# Autodesk Inventor assembly: Miniature_Steam_Engine
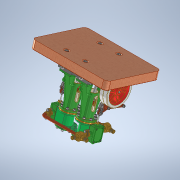
[picture p0: Inventor's stored thumbnail of the model, 180x180]
Saved by Autodesk Inventor 2020 (Build 240168000, 168)
## iProperties
Created: 2023-08-09
Part Number: Miniature_Steam_Engine
Document SubType Name: Assembly
Designer: ACER
Author: ACER
## Documents named in this file (59)
- D:\inventor\bt_tuluyen\ME\Miniature_Steam_Engine.iam
- D:\inventor\bt_tuluyen\ME\Stand_1.ipt
- D:\inventor\bt_tuluyen\ME\Base.ipt
- D:\inventor\bt_tuluyen\ME\Lower_Base_Bearing_Holder_4.ipt
- D:\inventor\bt_tuluyen\ME\Upper_Base_Bearing_Holder_7.ipt
- D:\inventor\bt_tuluyen\ME\Crankshaft.ipt
- D:\inventor\bt_tuluyen\ME\Upper_Base_Bearing_Holder2_8.ipt
- D:\inventor\bt_tuluyen\ME\Assembly_Eccentric.iam
- D:\inventor\bt_tuluyen\ME\Lower_Base_Bearing_Holder2_5.ipt
- D:\inventor\bt_tuluyen\ME\Welding_assembly_Standard.iam
- D:\inventor\bt_tuluyen\ME\Eccentric_rod.ipt
- D:\inventor\bt_tuluyen\ME\Flywhee_l.ipt
- D:\inventor\bt_tuluyen\ME\Bearing_Keeper_11.ipt
- D:\inventor\bt_tuluyen\ME\Conecting_Rod_12.ipt
- D:\inventor\bt_tuluyen\ME\Crankrod_13.ipt
- D:\inventor\bt_tuluyen\ME\Crosshead_14.ipt
- C:\Users\ACER\Documents\Inventor\Content Center Files\R2020\en-US\DIN 128\DIN 128 - A4.ipt
- C:\Users\ACER\Documents\Inventor\Content Center Files\R2020\en-US\DIN 912\DIN 912 - M4 x 0.7 x 30 x 20.ipt
- D:\inventor\bt_tuluyen\ME\Crankrod_Pin_15.ipt
- D:\inventor\bt_tuluyen\ME\Crankrod_Bolt_16.ipt
- D:\inventor\bt_tuluyen\ME\Cylinder_Packnut_18.ipt
- D:\inventor\bt_tuluyen\ME\Cylinder_cover_lower_19.ipt
- D:\inventor\bt_tuluyen\ME\Cylinder_left_.ipt
- D:\inventor\bt_tuluyen\ME\Cylinder_right_.ipt
- D:\inventor\bt_tuluyen\ME\Steam_Piston.ipt
- D:\inventor\bt_tuluyen\ME\Steam_Piston_Ring_.ipt
- D:\inventor\bt_tuluyen\ME\Steam_Piston_Rod_.ipt
- C:\Users\ACER\Documents\Inventor\Content Center Files\R2020\en-US\DIN 934\DIN 934 - M8 x 1.ipt
- D:\inventor\bt_tuluyen\ME\Cylinder_Packing_25.ipt
- D:\inventor\bt_tuluyen\ME\Upper_Cylinder_Cover_26.ipt
- D:\inventor\bt_tuluyen\ME\Assembly_Cylinder_piping_entry_.iam
- D:\inventor\bt_tuluyen\ME\Assembly_Cylinder_Piping_Exit_.iam
- D:\inventor\bt_tuluyen\ME\Valve_Plate_.ipt
- D:\inventor\bt_tuluyen\ME\Steamchest_.ipt
- D:\inventor\bt_tuluyen\ME\Valvel_Packnut_.ipt
- D:\inventor\bt_tuluyen\ME\Slide_Valve_.ipt
- D:\inventor\bt_tuluyen\ME\Side_Valve_Holder_.ipt
- D:\inventor\bt_tuluyen\ME\Steam_chest_slide_value_rod_.ipt
- D:\inventor\bt_tuluyen\ME\Steamchest_cover_.ipt
- D:\inventor\bt_tuluyen\ME\Reverse_Gear_Link_.ipt
- D:\inventor\bt_tuluyen\ME\Revert_Gear_Lever_God_.ipt
- D:\inventor\bt_tuluyen\ME\Reverse_gear_lever_.ipt
- D:\inventor\bt_tuluyen\ME\Revert_gear_level_link_pt.ipt
- D:\inventor\bt_tuluyen\ME\Revert_Gear_Drag_Link_.ipt
- D:\inventor\bt_tuluyen\ME\Cylinder_pipe_connector_42.ipt
- C:\Users\ACER\Documents\Inventor\Content Center Files\R2020\en-US\ISO 1207(1)\DIN EN ISO 1207 - M6 x 20.ipt
- C:\Users\ACER\Documents\Inventor\Content Center Files\R2020\en-US\DIN 128\DIN 128 - A6.ipt
- C:\Users\ACER\Documents\Inventor\Content Center Files\R2020\en-US\DIN 934\DIN 934 - M6 x 1.ipt
- C:\Users\ACER\Documents\Inventor\Content Center Files\R2020\en-US\ISO 1207(1)\DIN EN ISO 1207 - M6 x 45.ipt
- C:\Users\ACER\Documents\Inventor\Content Center Files\R2020\en-US\DIN 128\DIN 128 - A12.ipt
- C:\Users\ACER\Documents\Inventor\Content Center Files\R2020\en-US\DIN 912\DIN 912 - M12 x 1.75 x 55 x 36.ipt
- C:\Users\ACER\Documents\Inventor\Content Center Files\R2020\en-US\DIN 1587\DIN 1587 - M12 x 1.75.ipt
- C:\Users\ACER\Documents\Inventor\Content Center Files\R2020\en-US\DIN 125-1  A\DIN 125 - A 13.ipt
- C:\Users\ACER\Documents\Inventor\Content Center Files\R2020\en-US\DIN 912\DIN 912 - M6 x 1 x 12 x 9.5.ipt
- C:\Users\ACER\Documents\Inventor\Content Center Files\R2020\en-US\DIN 912\DIN 912 - M6 x 1 x 20 x 17.5.ipt
- C:\Users\ACER\Documents\Inventor\Content Center Files\R2020\en-US\DIN 933\DIN 933 - M6  x 20.ipt
- C:\Users\ACER\Documents\Inventor\Content Center Files\R2020\en-US\DIN 71412  A\DIN 71412 - AM 6 (coned short).ipt
- C:\Users\ACER\Documents\Inventor\Content Center Files\R2020\en-US\DIN 912\DIN 912 - M4 x 0.7 x 35 x 20.ipt
- C:\Users\ACER\Documents\Inventor\Content Center Files\R2020\en-US\DIN 916\DIN 916 - M4  x  5.ipt
## Components (313 placed, 58 different names)
1. Stand_1:1 — Mate:1, Mate:2, Mate:3, Mate:4, Mate:5, Angle:13, Insert:51, Insert:52, Insert:53, Insert:54
2. Base:1 — Mate:1, Mate:2, Mate:3, Mate:4, Mate:5, Mate:6, Mate:7, Mate:8, Mate:9, Mate:10, Mate:11, Mate:12, Mate:13, Mate:14, Mate:15, Flush:1, Mate:16, Mate:17, Flush:2, Mate:18, Mate:19, Mate:20, Mate:23, Mate:24, Mate:25, Mate:26, Mate:27, Mate:28, Mate:29, Mate:30, Mate:31, Mate:32, Angle:1, Angle:2, Mate:42, Mate:43, Mate:44, Mate:45, Mate:46, Mate:47, Mate:48, Mate:49, Mate:50, Angle:7, Mate:83, Insert:59, Insert:60, Insert:61, Insert:62
3. Upper_Base_Bearing_Holder_7:1 — Mate:11, Mate:12, Mate:13, Mate:35, Insert:128, Insert:129, Insert:146
4. Upper_Base_Bearing_Holder_7:2 — Mate:6, Mate:7, Mate:8, Mate:21, Angle:4, Insert:124, Insert:125, Insert:149
5. Crankshaft:1 — Mate:33, Mate:34, Mate:36, Mate:37, Flush:4, Mate:51, Mate:52, Mate:60, Mate:61, Mate:66, Mate:67, Mate:83, Angle:13, Mate:200, Mate:201
6. Upper_Base_Bearing_Holder2_8:1 — Mate:9, Mate:10, Mate:18, Flush:3, Insert:126, Insert:127, Insert:148
7. Assembly_Eccentric:1 [sub-assembly] — Mate:21, Angle:1, Mate:33, Mate:38, Flush:5, Mate:40, Flush:7, Mate:200, Mate:248, Flush:12
8. Lower_Base_Bearing_Holder_4:2 — Mate:14, Mate:15, Flush:1, Mate:34
9. Lower_Base_Bearing_Holder_4:3 — Mate:16, Mate:17, Flush:2
10. Lower_Base_Bearing_Holder2_5:1 — Mate:19, Mate:20, Flush:3
11. Welding_assembly_Standard:1 [sub-assembly] — Mate:23, Mate:24, Mate:25, Mate:26, Mate:27, Mate:91, Mate:106, Mate:107, Mate:194, Mate:202, Mate:212, Mate:216
12. Welding_assembly_Standard:2 [sub-assembly] — Mate:28, Mate:29, Mate:30, Mate:31, Mate:32, Mate:90, Mate:108, Mate:109, Mate:197, Mate:215, Insert:107, Insert:108, Insert:109, Insert:110, Insert:111
13. Assembly_Eccentric:2 [sub-assembly] — Mate:35, Angle:2, Mate:36, Flush:8, Mate:41, Mate:201, Mate:203, Flush:11, Mate:249, Flush:13
14. Eccentric_rod:1 — Mate:40, Flush:7, Mate:206, Insert:23, Insert:38, Insert:150
15. Eccentric_rod:2 — Mate:38, Flush:5, Angle:4, Angle:12, Angle:14, Mate:204, Insert:22, Insert:37, Insert:151
16. Eccentric_rod:3 — Mate:203, Flush:11, Mate:208, Mate:209, Insert:26, Insert:35, Insert:147
17. Eccentric_rod:4 — Flush:8, Mate:41, Angle:14, Mate:207, Angle:15, Insert:25, Insert:34, Insert:145
18. Flywhee_l:1 — Mate:37, Flush:4
19. Welding_assembly_Standard:3 [sub-assembly] — Mate:42, Mate:43, Mate:44, Mate:45, Mate:46, Insert:99, Insert:100, Insert:101, Insert:102, Insert:103, Insert:104, Insert:105, Insert:106, Insert:117, Insert:122, Insert:123, Insert:143
20. Welding_assembly_Standard:4 [sub-assembly] — Mate:47, Mate:48, Mate:49, Mate:50, Insert:112, Insert:113, Insert:114, Insert:118, Insert:119, Insert:120, Insert:121
21. Bearing_Keeper_11:1 — Mate:76, Mate:77, Mate:78, Mate:79, Mate:80, Mate:81, Mate:82
22. Bearing_Keeper_11:2 — Mate:53, Mate:54, Mate:55, Mate:72, Mate:73, Mate:74, Mate:75
23. Conecting_Rod_12:1 — Mate:52, Mate:56, Mate:57, Mate:58, Mate:59
24. Conecting_Rod_12:2 — Mate:51, Mate:53, Mate:54, Mate:55, Mate:58
25. Conecting_Rod_12:3 — Mate:61, Mate:62, Mate:63, Mate:64, Mate:65
26. Conecting_Rod_12:4 — Mate:60, Mate:62, Mate:76, Mate:77, Mate:78
27. Crankrod_13:1 — Mate:56, Mate:57, Mate:59, Mate:66, Angle:7, Mate:84, Mate:85, Mate:86, Insert:7
28. Crankrod_13:2 — Mate:63, Mate:64, Mate:65, Mate:67, Mate:87, Mate:88, Insert:9
29. Crosshead_14:1 — Mate:87, Mate:88, Mate:90, Mate:198
30. Crosshead_14:2 — Mate:84, Mate:85, Mate:86, Mate:91, Mate:196
31. DIN 128 A4:2 — Mate:81, Mate:82, Insert:4
32. DIN 128 A4:1 — Mate:79, Mate:80, Insert:5
33. DIN 128 A4:3 — Mate:72, Mate:74, Insert:3
34. DIN 128 A4:4 — Mate:73, Mate:75, Insert:6
35. DIN 912 - replaced by DIN EN ISO 4762 M4 x 30:1 — Insert:3
36. DIN 912 - replaced by DIN EN ISO 4762 M4 x 30:2 — Insert:6
37. DIN 912 - replaced by DIN EN ISO 4762 M4 x 30:3 — Insert:4
38. DIN 912 - replaced by DIN EN ISO 4762 M4 x 30:4 — Insert:5
39. Crankrod_Pin_15:1 — Insert:7, Insert:11
40. Crankrod_Pin_15:2 — Insert:9, Insert:12
41. Crankrod_Bolt_16:1 — Insert:12
42. Crankrod_Bolt_16:2 — Insert:11
43. Cylinder_Packnut_18:1 — Mate:105, Insert:16
44. Cylinder_Packnut_18:2 — Mate:104, Insert:15
45. Cylinder_cover_lower_19:1 — Insert:16, Mate:108, Mate:109, Mate:169, Mate:173
46. Cylinder_cover_lower_19:2 — Insert:15, Mate:106, Mate:107, Mate:171, Mate:172
47. Cylinder_left_:1 — Mate:170, Mate:171, Mate:172, Mate:178, Mate:179, Mate:180, Mate:181, Mate:182, Mate:186, Mate:187, Mate:188, Mate:190, Mate:194, Mate:231, Mate:235, Mate:236
48. Cylinder_right_:1 — Mate:168, Mate:169, Mate:173, Mate:174, Mate:175, Mate:176, Mate:177, Mate:183, Mate:184, Mate:185, Mate:191, Mate:192, Mate:197, Mate:229, Mate:237, Mate:238
49. Steam_Piston:1 — Mate:92, Mate:93, Mate:94, Mate:95, Mate:96, Insert:17, Mate:195
50. Steam_Piston:2 — Mate:98, Mate:99, Mate:100, Mate:101, Mate:103, Insert:18, Mate:199
51. Steam_Piston_Ring_:1 — Mate:94, Mate:95
52. Steam_Piston_Ring_:2 — Mate:92, Mate:93
53. Steam_Piston_Ring_:3 — Mate:98, Mate:99
54. Steam_Piston_Ring_:4 — Mate:100, Mate:101
55. Steam_Piston_Rod_:1 — Mate:96, Mate:104, Mate:170, Mate:195, Mate:196
56. Steam_Piston_Rod_:2 — Mate:103, Mate:105, Mate:168, Mate:198, Mate:199
57. DIN 934 - replaced by DIN EN 24032/28673/28674 M8 x 1:1 — Insert:17
58. DIN 934 - replaced by DIN EN 24032/28673/28674 M8 x 1:2 — Insert:18
59. Cylinder_Packing_25:1 — Mate:124, Mate:174, Mate:175
60. Cylinder_Packing_25:2 — Mate:126, Mate:180, Mate:181
61. Upper_Cylinder_Cover_26:1 — Mate:124, Mate:176, Mate:177, Insert:75, Insert:76, Insert:77, Insert:78, Insert:79, Insert:80, Insert:81, Insert:82
62. Upper_Cylinder_Cover_26:2 — Mate:126, Mate:178, Mate:179, Mate:182, Insert:67, Insert:68, Insert:69, Insert:70, Insert:71, Insert:72, Insert:73, Insert:74
63. Assembly_Cylinder_piping_entry_:1 [sub-assembly] — Mate:232, Mate:233, Mate:234
64. Assembly_Cylinder_Piping_Exit_:1 [sub-assembly] — Mate:229, Mate:231, Mate:239
65. Valve_Plate_:1 — Mate:138, Mate:152, Mate:186, Mate:187, Mate:188, Mate:189
66. Valve_Plate_:2 — Mate:141, Mate:149, Mate:183, Mate:184, Mate:185
67. Steamchest_:1 — Mate:138, Insert:19, Angle:10, Mate:159, Mate:160, Mate:189, Mate:190, Mate:232, Mate:234, Mate:241, Mate:242, Mate:245
68. Steamchest_:2 — Mate:141, Insert:20, Angle:9, Mate:155, Mate:157, Mate:158, Mate:164, Mate:165, Mate:166, Mate:167, Mate:191, Mate:192, Mate:233
69. Valvel_Packnut_:1 — Insert:20
70. Valvel_Packnut_:2 — Insert:19, Mate:145
71. Slide_Valve_:1 — Mate:152, Angle:10, Mate:154, Mate:159, Mate:160, Flush:9
72. Slide_Valve_:2 — Mate:149, Angle:9, Mate:150, Mate:157, Mate:158, Flush:10
73. Side_Valve_Holder_:1 — Mate:150, Mate:156, Flush:10
74. Side_Valve_Holder_:2 — Mate:153, Mate:154, Flush:9
75. Steam_chest_slide_value_rod_:1 — Mate:145, Mate:153, Angle:12, Mate:205, Insert:21, Insert:36
76. Steam_chest_slide_value_rod_:2 — Mate:155, Mate:156, Angle:15, Insert:24, Insert:33
77. Steamchest_cover_:1 — Mate:240, Mate:241, Mate:243, Mate:244, Mate:246, Insert:168, Mate:247
78. Steamchest_cover_:2 — Mate:164, Mate:165, Mate:166, Mate:167, Insert:156, Insert:157, Insert:158, Insert:159
79. Reverse_Gear_Link_:1 — Mate:204, Mate:205, Mate:206, Mate:217, Mate:218, Mate:220, Mate:221
80. Reverse_Gear_Link_:2 — Mate:207, Mate:208, Mate:209, Mate:223, Mate:224, Mate:226, Mate:227
81. Revert_Gear_Lever_God_:1 — Mate:202, Mate:210, Mate:211, Mate:213, Mate:214, Angle:17
82. Reverse_gear_lever_:1 — Mate:210, Mate:213, Angle:19, Mate:216, Insert:170, Insert:171
83. Revert_gear_level_link_pt:1 — Mate:211, Mate:212, Angle:17, Angle:19, Mate:219, Mate:222, Insert:169
84. Revert_gear_level_link_pt:2 — Mate:214, Mate:215, Mate:225, Mate:228, Insert:172
85. Revert_Gear_Drag_Link_:1 — Mate:217, Mate:218, Mate:219, Insert:47, Insert:48
86. Revert_Gear_Drag_Link_:2 — Mate:220, Mate:221, Mate:222, Insert:39, Insert:40
87. Revert_Gear_Drag_Link_:3 — Mate:226, Mate:227, Mate:228, Insert:49, Insert:50
88. Revert_Gear_Drag_Link_:4 — Mate:223, Mate:224, Mate:225, Insert:41, Insert:42
89. Cylinder_pipe_connector_42:1 — Mate:237, Mate:238
90. Cylinder_pipe_connector_42:2 — Mate:235, Mate:236, Mate:239
91. DIN EN ISO 1207 M6 x 20:1 — Insert:30
92. DIN EN ISO 1207 M6 x 20:2 — Insert:32
93. DIN EN ISO 1207 M6 x 20:3 — Insert:31
94. DIN EN ISO 1207 M6 x 20:4 — Insert:27
95. DIN EN ISO 1207 M6 x 20:5 — Insert:28
96. DIN EN ISO 1207 M6 x 20:6 — Insert:29
97. DIN 128 A6:1 — Insert:22, Insert:31
98. DIN 128 A6:2 — Insert:21, Insert:30
99. DIN 128 A6:3 — Insert:25, Insert:28
100. DIN 128 A6:4 — Insert:26, Insert:29
101. DIN 128 A6:5 — Insert:24, Insert:27
102. DIN 128 A6:6 — Insert:23, Insert:32
103. DIN 934 - replaced by DIN EN 24032/28673/28674 M6:1 — Insert:37
104. DIN 934 - replaced by DIN EN 24032/28673/28674 M6:2 — Insert:33
105. DIN 934 - replaced by DIN EN 24032/28673/28674 M6:3 — Insert:35
106. DIN 934 - replaced by DIN EN 24032/28673/28674 M6:4 — Insert:34
107. DIN 934 - replaced by DIN EN 24032/28673/28674 M6:5 — Insert:36
108. DIN 934 - replaced by DIN EN 24032/28673/28674 M6:6 — Insert:38
109. DIN EN ISO 1207 M6 x 45:1 — Insert:46
110. DIN EN ISO 1207 M6 x 45:2 — Insert:45
111. DIN EN ISO 1207 M6 x 45:3 — Insert:44
112. DIN EN ISO 1207 M6 x 45:4 — Insert:43
113. DIN 128 A6:7 — Insert:39, Insert:44
114. DIN 128 A6:8 — Insert:42, Insert:45
115. DIN 128 A6:9 — Insert:41, Insert:46
116. DIN 128 A6:10 — Insert:40, Insert:43
117. DIN 934 - replaced by DIN EN 24032/28673/28674 M6:7 — Insert:50
118. DIN 934 - replaced by DIN EN 24032/28673/28674 M6:8 — Insert:49
119. DIN 934 - replaced by DIN EN 24032/28673/28674 M6:9 — Insert:47
120. DIN 934 - replaced by DIN EN 24032/28673/28674 M6:10 — Insert:48
121. DIN 128 A12:1 — Insert:60, Insert:64
122. DIN 128 A12:2 — Insert:59, Insert:63
123. DIN 128 A12:3 — Insert:61, Insert:65
124. DIN 128 A12:4 — Insert:62, Insert:66
125. DIN 912 - replaced by DIN EN ISO 4762 M12 x 55:1 — Insert:55
126. DIN 912 - replaced by DIN EN ISO 4762 M12 x 55:2 — Insert:58
127. DIN 912 - replaced by DIN EN ISO 4762 M12 x 55:3 — Insert:57
128. DIN 912 - replaced by DIN EN ISO 4762 M12 x 55:4 — Insert:56
129. DIN 1587 M12 - SW18:1 — Insert:63
130. DIN 1587 M12 - SW18:2 — Insert:64
131. DIN 1587 M12 - SW18:3 — Insert:65
132. DIN 1587 M12 - SW18:4 — Insert:66
133. DIN 125-1 A A 13:1 — Insert:53, Insert:57
134. DIN 125-1 A A 13:2 — Insert:54, Insert:58
135. DIN 125-1 A A 13:3 — Insert:52, Insert:56
136. DIN 125-1 A A 13:4 — Insert:51, Insert:55
137. DIN 912 - replaced by DIN EN ISO 4762 M6 x 12:1 — Insert:85
138. DIN 912 - replaced by DIN EN ISO 4762 M6 x 12:2 — Insert:84
139. DIN 912 - replaced by DIN EN ISO 4762 M6 x 12:3 — Insert:86
140. DIN 912 - replaced by DIN EN ISO 4762 M6 x 12:4 — Insert:88
141. DIN 912 - replaced by DIN EN ISO 4762 M6 x 12:5 — Insert:91
142. DIN 912 - replaced by DIN EN ISO 4762 M6 x 12:6 — Insert:93
143. DIN 912 - replaced by DIN EN ISO 4762 M6 x 12:7 — Insert:95
144. DIN 912 - replaced by DIN EN ISO 4762 M6 x 12:8 — Insert:98
145. DIN 912 - replaced by DIN EN ISO 4762 M6 x 12:9 — Insert:90
146. DIN 912 - replaced by DIN EN ISO 4762 M6 x 12:10 — Insert:89
147. DIN 912 - replaced by DIN EN ISO 4762 M6 x 12:11 — Insert:83
148. DIN 912 - replaced by DIN EN ISO 4762 M6 x 12:12 — Insert:87
149. DIN 912 - replaced by DIN EN ISO 4762 M6 x 12:13 — Insert:92
150. DIN 912 - replaced by DIN EN ISO 4762 M6 x 12:14 — Insert:94
151. DIN 912 - replaced by DIN EN ISO 4762 M6 x 12:15 — Insert:96
152. DIN 912 - replaced by DIN EN ISO 4762 M6 x 12:16 — Insert:97
153. DIN 128 A6:11 — Insert:67, Insert:84
154. DIN 128 A6:12 — Insert:68, Insert:83
155. DIN 128 A6:13 — Insert:69, Insert:86
156. DIN 128 A6:14 — Insert:70, Insert:87
157. DIN 128 A6:15 — Insert:71, Insert:88
158. DIN 128 A6:16 — Insert:72, Insert:89
159. DIN 128 A6:17 — Insert:73, Insert:90
160. DIN 128 A6:18 — Insert:74, Insert:85
161. DIN 128 A6:19 — Insert:77, Insert:93
162. DIN 128 A6:20 — Insert:76, Insert:95
163. DIN 128 A6:21 — Insert:79, Insert:91
164. DIN 128 A6:22 — Insert:78, Insert:92
165. DIN 128 A6:23 — Insert:80, Insert:98
166. DIN 128 A6:24 — Insert:82, Insert:96
167. DIN 128 A6:25 — Insert:81, Insert:97
168. DIN 128 A6:26 — Insert:75, Insert:94
169. DIN 128 A6:27 — Insert:113
170. DIN 128 A6:28 — Insert:114
171. DIN 128 A6:29 — Insert:112
172. DIN 128 A6:30 — Insert:111
173. DIN 128 A6:31 — Insert:110, Insert:116
174. DIN 128 A6:32 — Insert:109
175. DIN 128 A6:33 — Insert:108
176. DIN 128 A6:34 — Insert:107
177. DIN 128 A6:35 — Insert:106
178. DIN 128 A6:36 — Insert:104
179. DIN 128 A6:37 — Insert:105
180. DIN 128 A6:38 — Insert:103
181. DIN 128 A6:39 — Insert:102
182. DIN 128 A6:40 — Insert:101
183. DIN 128 A6:41 — Insert:99
184. DIN 128 A6:42 — Insert:100, Insert:115
185. DIN 933 - replaced by DIN EN 24017 M6  x 20:1 — Insert:142
186. DIN 933 - replaced by DIN EN 24017 M6  x 20:2 — Insert:141
187. DIN 933 - replaced by DIN EN 24017 M6  x 20:3 — Insert:140
188. DIN 933 - replaced by DIN EN 24017 M6  x 20:4 — Insert:144
189. DIN 933 - replaced by DIN EN 24017 M6  x 20:5 — Insert:139
190. DIN 933 - replaced by DIN EN 24017 M6  x 20:6 — Insert:138
191. DIN 933 - replaced by DIN EN 24017 M6  x 20:7 — Insert:131
192. DIN 933 - replaced by DIN EN 24017 M6  x 20:8 — Insert:130
193. DIN 933 - replaced by DIN EN 24017 M6  x 20:9 — Insert:136
194. DIN 933 - replaced by DIN EN 24017 M6  x 20:10 — Insert:137
195. DIN 933 - replaced by DIN EN 24017 M6  x 20:11 — Insert:135
196. DIN 933 - replaced by DIN EN 24017 M6  x 20:12 — Insert:132
197. DIN 933 - replaced by DIN EN 24017 M6  x 20:13 — Insert:134
198. DIN 933 - replaced by DIN EN 24017 M6  x 20:14 — Insert:133
199. DIN 128 A6:43 — Insert:118, Insert:141
200. DIN 128 A6:44 — Insert:143, Insert:144
201. DIN 128 A6:45 — Insert:119, Insert:142
202. DIN 128 A6:46 — Insert:117, Insert:140
203. DIN 128 A6:47 — Insert:121, Insert:133
204. DIN 128 A6:48 — Insert:120, Insert:132
205. DIN 128 A6:49 — Insert:123, Insert:130
206. DIN 128 A6:50 — Insert:122, Insert:131
207. DIN 128 A6:51 — Insert:125, Insert:137
208. DIN 128 A6:52 — Insert:124, Insert:136
209. DIN 128 A6:53 — Insert:129, Insert:135
210. DIN 128 A6:54 — Insert:126, Insert:139
211. DIN 128 A6:55 — Insert:128, Insert:138
212. DIN 128 A6:56 — Insert:127, Insert:134
213. DIN 71412 A AM 6 (coned short):1 — Insert:146
214. DIN 71412 A AM 6 (coned short):2 — Insert:148
215. DIN 71412 A AM 6 (coned short):3 — Insert:145
216. DIN 71412 A AM 6 (coned short):4 — Insert:147
217. DIN 71412 A AM 6 (coned short):5 — Insert:150
218. DIN 71412 A AM 6 (coned short):6 — Insert:149
219. DIN 71412 A AM 6 (coned short):7 — Insert:151
220. DIN 912 - replaced by DIN EN ISO 4762 M4 x 35:1 — Insert:166, Mate:244, Mate:245
221. DIN 912 - replaced by DIN EN ISO 4762 M4 x 35:2 — Insert:167
222. DIN 912 - replaced by DIN EN ISO 4762 M4 x 35:3 — Insert:165
223. DIN 912 - replaced by DIN EN ISO 4762 M4 x 35:4 — Insert:164, Mate:240, Mate:242
224. DIN 912 - replaced by DIN EN ISO 4762 M4 x 35:5 — Insert:162
225. DIN 912 - replaced by DIN EN ISO 4762 M4 x 35:6 — Insert:163
226. DIN 912 - replaced by DIN EN ISO 4762 M4 x 35:7 — Insert:161
227. DIN 912 - replaced by DIN EN ISO 4762 M4 x 35:8 — Insert:160
228. DIN 128 A4:5 — Insert:159, Insert:162
229. DIN 128 A4:6 — Insert:156, Insert:160
230. DIN 128 A4:7 — Insert:158, Insert:163
231. DIN 128 A4:8 — Insert:157, Insert:161
232. DIN 128 A4:9 — Insert:167, Insert:168
233. DIN 128 A4:10 — Insert:165, Mate:247
234. DIN 128 A4:11 — Insert:166, Mate:246
235. DIN 128 A4:12 — Insert:164, Mate:243
236. DIN 916 M4  x  5:1 — Mate:249, Flush:13
237. DIN 916 M4  x  5:2 — Insert:172
238. DIN 916 M4  x  5:3 — Insert:169
239. DIN 916 M4  x  5:4 — Insert:171
240. DIN 916 M4  x  5:5 — Mate:248, Flush:12
241. DIN 916 M4  x  5:6 — Insert:170
242. DIN 912 - replaced by DIN EN ISO 4762 M6 x 20:1 — Insert:116
243. DIN 912 - replaced by DIN EN ISO 4762 M6 x 20:80
244. DIN 912 - replaced by DIN EN ISO 4762 M6 x 20:81
245. DIN 912 - replaced by DIN EN ISO 4762 M6 x 20:82
246. DIN 912 - replaced by DIN EN ISO 4762 M6 x 20:83
247. DIN 912 - replaced by DIN EN ISO 4762 M6 x 20:84
248. DIN 912 - replaced by DIN EN ISO 4762 M6 x 20:85
249. DIN 912 - replaced by DIN EN ISO 4762 M6 x 20:86
250. DIN 912 - replaced by DIN EN ISO 4762 M6 x 20:13 — Insert:115
251. DIN 912 - replaced by DIN EN ISO 4762 M6 x 20:17
252. DIN 912 - replaced by DIN EN ISO 4762 M6 x 20:18
253. DIN 912 - replaced by DIN EN ISO 4762 M6 x 20:19
254. DIN 912 - replaced by DIN EN ISO 4762 M6 x 20:20
255. DIN 912 - replaced by DIN EN ISO 4762 M6 x 20:21
256. DIN 912 - replaced by DIN EN ISO 4762 M6 x 20:22
257. DIN 912 - replaced by DIN EN ISO 4762 M6 x 20:23
258. DIN 912 - replaced by DIN EN ISO 4762 M6 x 20:24
259. DIN 912 - replaced by DIN EN ISO 4762 M6 x 20:25
260. DIN 912 - replaced by DIN EN ISO 4762 M6 x 20:26
261. DIN 912 - replaced by DIN EN ISO 4762 M6 x 20:27
262. DIN 912 - replaced by DIN EN ISO 4762 M6 x 20:28
263. DIN 912 - replaced by DIN EN ISO 4762 M6 x 20:29
264. DIN 912 - replaced by DIN EN ISO 4762 M6 x 20:30
265. DIN 912 - replaced by DIN EN ISO 4762 M6 x 20:31
266. DIN 912 - replaced by DIN EN ISO 4762 M6 x 20:32
267. DIN 912 - replaced by DIN EN ISO 4762 M6 x 20:33
268. DIN 912 - replaced by DIN EN ISO 4762 M6 x 20:34
269. DIN 912 - replaced by DIN EN ISO 4762 M6 x 20:35
270. DIN 912 - replaced by DIN EN ISO 4762 M6 x 20:36
271. DIN 912 - replaced by DIN EN ISO 4762 M6 x 20:37
272. DIN 912 - replaced by DIN EN ISO 4762 M6 x 20:38
273. DIN 912 - replaced by DIN EN ISO 4762 M6 x 20:39
274. DIN 912 - replaced by DIN EN ISO 4762 M6 x 20:40
275. DIN 912 - replaced by DIN EN ISO 4762 M6 x 20:41
276. DIN 912 - replaced by DIN EN ISO 4762 M6 x 20:42
277. DIN 912 - replaced by DIN EN ISO 4762 M6 x 20:43
278. DIN 912 - replaced by DIN EN ISO 4762 M6 x 20:44
279. DIN 912 - replaced by DIN EN ISO 4762 M6 x 20:45
280. DIN 912 - replaced by DIN EN ISO 4762 M6 x 20:46
281. DIN 912 - replaced by DIN EN ISO 4762 M6 x 20:47
282. DIN 912 - replaced by DIN EN ISO 4762 M6 x 20:48
283. DIN 912 - replaced by DIN EN ISO 4762 M6 x 20:49
284. DIN 912 - replaced by DIN EN ISO 4762 M6 x 20:50
285. DIN 912 - replaced by DIN EN ISO 4762 M6 x 20:51
286. DIN 912 - replaced by DIN EN ISO 4762 M6 x 20:52
287. DIN 912 - replaced by DIN EN ISO 4762 M6 x 20:53
288. DIN 912 - replaced by DIN EN ISO 4762 M6 x 20:54
289. DIN 912 - replaced by DIN EN ISO 4762 M6 x 20:55
290. DIN 912 - replaced by DIN EN ISO 4762 M6 x 20:56
291. DIN 912 - replaced by DIN EN ISO 4762 M6 x 20:57
292. DIN 912 - replaced by DIN EN ISO 4762 M6 x 20:58
293. DIN 912 - replaced by DIN EN ISO 4762 M6 x 20:59
294. DIN 912 - replaced by DIN EN ISO 4762 M6 x 20:60
295. DIN 912 - replaced by DIN EN ISO 4762 M6 x 20:61
296. DIN 912 - replaced by DIN EN ISO 4762 M6 x 20:62
297. DIN 912 - replaced by DIN EN ISO 4762 M6 x 20:63
298. DIN 912 - replaced by DIN EN ISO 4762 M6 x 20:64
299. DIN 912 - replaced by DIN EN ISO 4762 M6 x 20:65
300. DIN 912 - replaced by DIN EN ISO 4762 M6 x 20:66
301. DIN 912 - replaced by DIN EN ISO 4762 M6 x 20:67
302. DIN 912 - replaced by DIN EN ISO 4762 M6 x 20:68
303. DIN 912 - replaced by DIN EN ISO 4762 M6 x 20:69
304. DIN 912 - replaced by DIN EN ISO 4762 M6 x 20:70
305. DIN 912 - replaced by DIN EN ISO 4762 M6 x 20:71
306. DIN 912 - replaced by DIN EN ISO 4762 M6 x 20:72
307. DIN 912 - replaced by DIN EN ISO 4762 M6 x 20:73
308. DIN 912 - replaced by DIN EN ISO 4762 M6 x 20:74
309. DIN 912 - replaced by DIN EN ISO 4762 M6 x 20:75
310. DIN 912 - replaced by DIN EN ISO 4762 M6 x 20:76
311. DIN 912 - replaced by DIN EN ISO 4762 M6 x 20:77
312. DIN 912 - replaced by DIN EN ISO 4762 M6 x 20:78
313. DIN 912 - replaced by DIN EN ISO 4762 M6 x 20:79
## Component patterns: (8 elements), (8 elements, first: DIN 912 - replaced by DIN EN ISO 4762 M6 x 20:1), (8 elements, first: DIN 912 - replaced by DIN EN ISO 4762 M6 x 20:13), Component Pattern 1:2 (8 elements), Component Pattern 1:3 (8 elements), Component Pattern 1:4 (8 elements), Component Pattern 1:5 (8 elements), Component Pattern 1:6 (8 elements), Component Pattern 1:7 (8 elements), Component Pattern 1:8 (8 elements)
## Relationships (386: Mate 200, Insert 162, Flush 12, Angle 12)
- Mate:1: Stand_1:1 ↔ Base:1
- Mate:2: Stand_1:1 ↔ Base:1
- Mate:3: Stand_1:1 ↔ Base:1
- Mate:4: Stand_1:1 ↔ Base:1
- Mate:5: Stand_1:1 ↔ Base:1
- Mate:6: Base:1 ↔ Upper_Base_Bearing_Holder_7:2
- Mate:7: Base:1 ↔ Upper_Base_Bearing_Holder_7:2
- Mate:8: Base:1 ↔ Upper_Base_Bearing_Holder_7:2
- Mate:9: Base:1 ↔ Upper_Base_Bearing_Holder2_8:1
- Mate:10: Base:1 ↔ Upper_Base_Bearing_Holder2_8:1
- Mate:11: Base:1 ↔ Upper_Base_Bearing_Holder_7:1
- Mate:12: Base:1 ↔ Upper_Base_Bearing_Holder_7:1
- Mate:13: Base:1 ↔ Upper_Base_Bearing_Holder_7:1
- Mate:14: Base:1 ↔ Lower_Base_Bearing_Holder_4:2
- Mate:15: Base:1 ↔ Lower_Base_Bearing_Holder_4:2
- Flush:1: Base:1 ↔ Lower_Base_Bearing_Holder_4:2
- Mate:16: Base:1 ↔ Lower_Base_Bearing_Holder_4:3
- Mate:17: Base:1 ↔ Lower_Base_Bearing_Holder_4:3
- Flush:2: Base:1 ↔ Lower_Base_Bearing_Holder_4:3
- Mate:18: Base:1 ↔ Upper_Base_Bearing_Holder2_8:1
- Mate:19: Base:1 ↔ Lower_Base_Bearing_Holder2_5:1
- Mate:20: Base:1 ↔ Lower_Base_Bearing_Holder2_5:1
- Flush:3: Upper_Base_Bearing_Holder2_8:1 ↔ Lower_Base_Bearing_Holder2_5:1
- Mate:21: Upper_Base_Bearing_Holder_7:2 ↔ Assembly_Eccentric:1
- Mate:23: Base:1 ↔ Welding_assembly_Standard:1
- Mate:24: Base:1 ↔ Welding_assembly_Standard:1
- Mate:25: Base:1 ↔ Welding_assembly_Standard:1
- Mate:26: Base:1 ↔ Welding_assembly_Standard:1
- Mate:27: Base:1 ↔ Welding_assembly_Standard:1
- Mate:28: Base:1 ↔ Welding_assembly_Standard:2
- Mate:29: Base:1 ↔ Welding_assembly_Standard:2
- Mate:30: Base:1 ↔ Welding_assembly_Standard:2
- Mate:31: Base:1 ↔ Welding_assembly_Standard:2
- Mate:32: Base:1 ↔ Welding_assembly_Standard:2
- Angle:1 (180 deg): Base:1 ↔ Assembly_Eccentric:1
- Mate:33: Crankshaft:1 ↔ Assembly_Eccentric:1
- Mate:34: Crankshaft:1 ↔ Lower_Base_Bearing_Holder_4:2
- Mate:35: Upper_Base_Bearing_Holder_7:1 ↔ Assembly_Eccentric:2
- Angle:2 (0 deg): Base:1 ↔ Assembly_Eccentric:2
- Mate:36: Crankshaft:1 ↔ Assembly_Eccentric:2
- Mate:37: Crankshaft:1 ↔ Flywhee_l:1
- Flush:4: Crankshaft:1 ↔ Flywhee_l:1
- Mate:38: Assembly_Eccentric:1 ↔ Eccentric_rod:2
- Flush:5: Assembly_Eccentric:1 ↔ Eccentric_rod:2
- Angle:4 (0 deg): Upper_Base_Bearing_Holder_7:2 ↔ Eccentric_rod:2
- Mate:40: Assembly_Eccentric:1 ↔ Eccentric_rod:1
- Flush:7: Assembly_Eccentric:1 ↔ Eccentric_rod:1
- Flush:8: Assembly_Eccentric:2 ↔ Eccentric_rod:4
- Mate:41: Assembly_Eccentric:2 ↔ Eccentric_rod:4
- Mate:42: Base:1 ↔ Welding_assembly_Standard:3
- Mate:43: Base:1 ↔ Welding_assembly_Standard:3
- Mate:44: Base:1 ↔ Welding_assembly_Standard:3
- Mate:45: Base:1 ↔ Welding_assembly_Standard:3
- Mate:46: Base:1 ↔ Welding_assembly_Standard:3
- Mate:47: Base:1 ↔ Welding_assembly_Standard:4
- Mate:48: Base:1 ↔ Welding_assembly_Standard:4
- Mate:49: Base:1 ↔ Welding_assembly_Standard:4
- Mate:50: Base:1 ↔ Welding_assembly_Standard:4
- Mate:51: Crankshaft:1 ↔ Conecting_Rod_12:2
- Mate:52: Crankshaft:1 ↔ Conecting_Rod_12:1
- Mate:53: Bearing_Keeper_11:2 ↔ Conecting_Rod_12:2
- Mate:54: Bearing_Keeper_11:2 ↔ Conecting_Rod_12:2
- Mate:55: Bearing_Keeper_11:2 ↔ Conecting_Rod_12:2
- Mate:56: Conecting_Rod_12:1 ↔ Crankrod_13:1
- Mate:57: Conecting_Rod_12:1 ↔ Crankrod_13:1
- Mate:58: Conecting_Rod_12:1 ↔ Conecting_Rod_12:2
- Mate:59: Conecting_Rod_12:1 ↔ Crankrod_13:1
- Mate:60: Crankshaft:1 ↔ Conecting_Rod_12:4
- Mate:61: Crankshaft:1 ↔ Conecting_Rod_12:3
- Mate:62: Conecting_Rod_12:3 ↔ Conecting_Rod_12:4
- Mate:63: Conecting_Rod_12:3 ↔ Crankrod_13:2
- Mate:64: Conecting_Rod_12:3 ↔ Crankrod_13:2
- Mate:65: Conecting_Rod_12:3 ↔ Crankrod_13:2
- Mate:66 (1.5 mm): Crankshaft:1 ↔ Crankrod_13:1
- Mate:67 (1.5 mm): Crankshaft:1 ↔ Crankrod_13:2
- Mate:72: Bearing_Keeper_11:2 ↔ DIN 128 A4:3
- Mate:73: Bearing_Keeper_11:2 ↔ DIN 128 A4:4
- Mate:74: Bearing_Keeper_11:2 ↔ DIN 128 A4:3
- Mate:75: Bearing_Keeper_11:2 ↔ DIN 128 A4:4
- Insert:3: DIN 128 A4:3 ↔ DIN 912 - replaced by DIN EN ISO 4762 M4 x 30:1
- Mate:76: Bearing_Keeper_11:1 ↔ Conecting_Rod_12:4
- Mate:77: Bearing_Keeper_11:1 ↔ Conecting_Rod_12:4
- Mate:78: Bearing_Keeper_11:1 ↔ Conecting_Rod_12:4
- Mate:79: Bearing_Keeper_11:1 ↔ DIN 128 A4:1
- Mate:80: Bearing_Keeper_11:1 ↔ DIN 128 A4:1
- Mate:81: Bearing_Keeper_11:1 ↔ DIN 128 A4:2
- Mate:82: Bearing_Keeper_11:1 ↔ DIN 128 A4:2
- Insert:4: DIN 128 A4:2 ↔ DIN 912 - replaced by DIN EN ISO 4762 M4 x 30:3
- Insert:5: DIN 128 A4:1 ↔ DIN 912 - replaced by DIN EN ISO 4762 M4 x 30:4
- Insert:6: DIN 128 A4:4 ↔ DIN 912 - replaced by DIN EN ISO 4762 M4 x 30:2
- Angle:7 (0 deg): Base:1 ↔ Crankrod_13:1
- Mate:83 (4 mm): Base:1 ↔ Crankshaft:1
- Mate:84: Crankrod_13:1 ↔ Crosshead_14:2
- Mate:85: Crankrod_13:1 ↔ Crosshead_14:2
- Mate:86: Crankrod_13:1 ↔ Crosshead_14:2
- Insert:7: Crankrod_13:1 ↔ Crankrod_Pin_15:1
- Mate:87: Crankrod_13:2 ↔ Crosshead_14:1
- Mate:88: Crankrod_13:2 ↔ Crosshead_14:1
- Insert:9: Crankrod_13:2 ↔ Crankrod_Pin_15:2
- Mate:90: Welding_assembly_Standard:2 ↔ Crosshead_14:1
- Insert:11: Crankrod_Pin_15:1 ↔ Crankrod_Bolt_16:2
- Insert:12: Crankrod_Pin_15:2 ↔ Crankrod_Bolt_16:1
- Mate:91: Welding_assembly_Standard:1 ↔ Crosshead_14:2
- Mate:92: Steam_Piston:1 ↔ Steam_Piston_Ring_:2
- Mate:93: Steam_Piston:1 ↔ Steam_Piston_Ring_:2
- Mate:94: Steam_Piston:1 ↔ Steam_Piston_Ring_:1
- Mate:95: Steam_Piston:1 ↔ Steam_Piston_Ring_:1
- Mate:96: Steam_Piston:1 ↔ Steam_Piston_Rod_:1
- Mate:98: Steam_Piston:2 ↔ Steam_Piston_Ring_:3
- Mate:99: Steam_Piston:2 ↔ Steam_Piston_Ring_:3
- Mate:100: Steam_Piston:2 ↔ Steam_Piston_Ring_:4
- Mate:101: Steam_Piston:2 ↔ Steam_Piston_Ring_:4
- Mate:103: Steam_Piston:2 ↔ Steam_Piston_Rod_:2
- Mate:104: Cylinder_Packnut_18:2 ↔ Steam_Piston_Rod_:1
- Mate:105: Cylinder_Packnut_18:1 ↔ Steam_Piston_Rod_:2
- Insert:15: Cylinder_Packnut_18:2 ↔ Cylinder_cover_lower_19:2
- Insert:16: Cylinder_Packnut_18:1 ↔ Cylinder_cover_lower_19:1
- Mate:106: Welding_assembly_Standard:1 ↔ Cylinder_cover_lower_19:2
- Mate:107: Welding_assembly_Standard:1 ↔ Cylinder_cover_lower_19:2
- Mate:108: Welding_assembly_Standard:2 ↔ Cylinder_cover_lower_19:1
- Mate:109: Welding_assembly_Standard:2 ↔ Cylinder_cover_lower_19:1
- Insert:17: Steam_Piston:1 ↔ DIN 934 - replaced by DIN EN 24032/28673/28674 M8 x 1:1
- Insert:18: Steam_Piston:2 ↔ DIN 934 - replaced by DIN EN 24032/28673/28674 M8 x 1:2
- Mate:124: Cylinder_Packing_25:1 ↔ Upper_Cylinder_Cover_26:1
- Mate:126: Cylinder_Packing_25:2 ↔ Upper_Cylinder_Cover_26:2
- Mate:138: Valve_Plate_:1 ↔ Steamchest_:1
- Mate:141: Valve_Plate_:2 ↔ Steamchest_:2
- Insert:19: Steamchest_:1 ↔ Valvel_Packnut_:2
- Insert:20: Steamchest_:2 ↔ Valvel_Packnut_:1
- Mate:145: Valvel_Packnut_:2 ↔ Steam_chest_slide_value_rod_:1
- Mate:149: Valve_Plate_:2 ↔ Slide_Valve_:2
- Angle:9 (0 deg): Steamchest_:2 ↔ Slide_Valve_:2
- Mate:150: Slide_Valve_:2 ↔ Side_Valve_Holder_:1
- Mate:152: Valve_Plate_:1 ↔ Slide_Valve_:1
- Angle:10 (0 deg): Steamchest_:1 ↔ Slide_Valve_:1
- Mate:153: Side_Valve_Holder_:2 ↔ Steam_chest_slide_value_rod_:1
- Mate:154: Slide_Valve_:1 ↔ Side_Valve_Holder_:2
- Mate:155: Steamchest_:2 ↔ Steam_chest_slide_value_rod_:2
- Mate:156: Side_Valve_Holder_:1 ↔ Steam_chest_slide_value_rod_:2
- Mate:157 (6 mm): Steamchest_:2 ↔ Slide_Valve_:2
- Mate:158 (10.5 mm): Steamchest_:2 ↔ Slide_Valve_:2
- Mate:159 (6 mm): Steamchest_:1 ↔ Slide_Valve_:1
- Mate:160 (10.5 mm): Steamchest_:1 ↔ Slide_Valve_:1
- Angle:12 (0 deg): Eccentric_rod:2 ↔ Steam_chest_slide_value_rod_:1
- Mate:164: Steamchest_:2 ↔ Steamchest_cover_:2
- Mate:165: Steamchest_:2 ↔ Steamchest_cover_:2
- Mate:166: Steamchest_:2 ↔ Steamchest_cover_:2
- Mate:167: Steamchest_:2 ↔ Steamchest_cover_:2
- Mate:168: Cylinder_right_:1 ↔ Steam_Piston_Rod_:2
- Mate:169: Cylinder_cover_lower_19:1 ↔ Cylinder_right_:1
- Mate:170: Cylinder_left_:1 ↔ Steam_Piston_Rod_:1
- Mate:171: Cylinder_cover_lower_19:2 ↔ Cylinder_left_:1
- Mate:172: Cylinder_cover_lower_19:2 ↔ Cylinder_left_:1
- Mate:173: Cylinder_cover_lower_19:1 ↔ Cylinder_right_:1
- Mate:174: Cylinder_right_:1 ↔ Cylinder_Packing_25:1
- Mate:175: Cylinder_right_:1 ↔ Cylinder_Packing_25:1
- Mate:176: Cylinder_right_:1 ↔ Upper_Cylinder_Cover_26:1
- Mate:177: Cylinder_right_:1 ↔ Upper_Cylinder_Cover_26:1
- Mate:178: Cylinder_left_:1 ↔ Upper_Cylinder_Cover_26:2
- Mate:179: Cylinder_left_:1 ↔ Upper_Cylinder_Cover_26:2
- Mate:180: Cylinder_left_:1 ↔ Cylinder_Packing_25:2
- Mate:181: Cylinder_left_:1 ↔ Cylinder_Packing_25:2
- Mate:182: Cylinder_left_:1 ↔ Upper_Cylinder_Cover_26:2
- Mate:183: Cylinder_right_:1 ↔ Valve_Plate_:2
- Mate:184: Cylinder_right_:1 ↔ Valve_Plate_:2
- Mate:185: Cylinder_right_:1 ↔ Valve_Plate_:2
- Mate:186: Cylinder_left_:1 ↔ Valve_Plate_:1
- Mate:187: Cylinder_left_:1 ↔ Valve_Plate_:1
- Mate:188: Cylinder_left_:1 ↔ Valve_Plate_:1
- Mate:189: Valve_Plate_:1 ↔ Steamchest_:1
- Mate:190: Cylinder_left_:1 ↔ Steamchest_:1
- Mate:191: Cylinder_right_:1 ↔ Steamchest_:2
- Mate:192: Cylinder_right_:1 ↔ Steamchest_:2
- Flush:9 (4.5 mm): Slide_Valve_:1 ↔ Side_Valve_Holder_:2
- Flush:10 (4.5 mm): Slide_Valve_:2 ↔ Side_Valve_Holder_:1
- Mate:194: Welding_assembly_Standard:1 ↔ Cylinder_left_:1
- Mate:195: Steam_Piston:1 ↔ Steam_Piston_Rod_:1
- Mate:196 (2 mm): Crosshead_14:2 ↔ Steam_Piston_Rod_:1
- Mate:197: Welding_assembly_Standard:2 ↔ Cylinder_right_:1
- Mate:198 (2 mm): Crosshead_14:1 ↔ Steam_Piston_Rod_:2
- Mate:199: Steam_Piston:2 ↔ Steam_Piston_Rod_:2
- Angle:13 (180 deg): Stand_1:1 ↔ Crankshaft:1
- Mate:200: Crankshaft:1 ↔ Assembly_Eccentric:1
- Mate:201: Crankshaft:1 ↔ Assembly_Eccentric:2
- Angle:14 (0 deg): Eccentric_rod:2 ↔ Eccentric_rod:4
- Mate:202: Welding_assembly_Standard:1 ↔ Revert_Gear_Lever_God_:1
- Mate:203: Assembly_Eccentric:2 ↔ Eccentric_rod:3
- Flush:11: Assembly_Eccentric:2 ↔ Eccentric_rod:3
- Mate:204: Eccentric_rod:2 ↔ Reverse_Gear_Link_:1
- Mate:205 (0.5 mm): Steam_chest_slide_value_rod_:1 ↔ Reverse_Gear_Link_:1
- Mate:206: Eccentric_rod:1 ↔ Reverse_Gear_Link_:1
- Mate:207: Eccentric_rod:4 ↔ Reverse_Gear_Link_:2
- Mate:208: Eccentric_rod:3 ↔ Reverse_Gear_Link_:2
- Mate:209 (0.5 mm): Eccentric_rod:3 ↔ Reverse_Gear_Link_:2
- Angle:15 (0 deg): Eccentric_rod:4 ↔ Steam_chest_slide_value_rod_:2
- Mate:210: Revert_Gear_Lever_God_:1 ↔ Reverse_gear_lever_:1
- Mate:211: Revert_Gear_Lever_God_:1 ↔ Revert_gear_level_link_pt:1
- Mate:212: Welding_assembly_Standard:1 ↔ Revert_gear_level_link_pt:1
- Mate:213: Revert_Gear_Lever_God_:1 ↔ Reverse_gear_lever_:1
- Mate:214: Revert_Gear_Lever_God_:1 ↔ Revert_gear_level_link_pt:2
- Mate:215: Welding_assembly_Standard:2 ↔ Revert_gear_level_link_pt:2
- Angle:17 (0 deg): Revert_Gear_Lever_God_:1 ↔ Revert_gear_level_link_pt:1
- Angle:19 (0 deg): Reverse_gear_lever_:1 ↔ Revert_gear_level_link_pt:1
- Mate:216 (25 mm): Welding_assembly_Standard:1 ↔ Reverse_gear_lever_:1
- Mate:217: Reverse_Gear_Link_:1 ↔ Revert_Gear_Drag_Link_:1
- Mate:218: Reverse_Gear_Link_:1 ↔ Revert_Gear_Drag_Link_:1
- Mate:219: Revert_gear_level_link_pt:1 ↔ Revert_Gear_Drag_Link_:1
- Mate:220: Reverse_Gear_Link_:1 ↔ Revert_Gear_Drag_Link_:2
- Mate:221: Reverse_Gear_Link_:1 ↔ Revert_Gear_Drag_Link_:2
- Mate:222: Revert_gear_level_link_pt:1 ↔ Revert_Gear_Drag_Link_:2
- Mate:223: Reverse_Gear_Link_:2 ↔ Revert_Gear_Drag_Link_:4
- Mate:224: Reverse_Gear_Link_:2 ↔ Revert_Gear_Drag_Link_:4
- Mate:225: Revert_gear_level_link_pt:2 ↔ Revert_Gear_Drag_Link_:4
- Mate:226: Reverse_Gear_Link_:2 ↔ Revert_Gear_Drag_Link_:3
- Mate:227: Reverse_Gear_Link_:2 ↔ Revert_Gear_Drag_Link_:3
- Mate:228: Revert_gear_level_link_pt:2 ↔ Revert_Gear_Drag_Link_:3
- Mate:229: Cylinder_right_:1 ↔ Assembly_Cylinder_Piping_Exit_:1
- Mate:231: Cylinder_left_:1 ↔ Assembly_Cylinder_Piping_Exit_:1
- Mate:232: Assembly_Cylinder_piping_entry_:1 ↔ Steamchest_:1
- Mate:233: Assembly_Cylinder_piping_entry_:1 ↔ Steamchest_:2
- Mate:234: Assembly_Cylinder_piping_entry_:1 ↔ Steamchest_:1
- Mate:235: Cylinder_left_:1 ↔ Cylinder_pipe_connector_42:2
- Mate:236: Cylinder_left_:1 ↔ Cylinder_pipe_connector_42:2
- Mate:237: Cylinder_right_:1 ↔ Cylinder_pipe_connector_42:1
- Mate:238: Cylinder_right_:1 ↔ Cylinder_pipe_connector_42:1
- Mate:239: Assembly_Cylinder_Piping_Exit_:1 ↔ Cylinder_pipe_connector_42:2
- Insert:21: Steam_chest_slide_value_rod_:1 ↔ DIN 128 A6:2
- Insert:22: Eccentric_rod:2 ↔ DIN 128 A6:1
- Insert:23: Eccentric_rod:1 ↔ DIN 128 A6:6
- Insert:24: Steam_chest_slide_value_rod_:2 ↔ DIN 128 A6:5
- Insert:25: Eccentric_rod:4 ↔ DIN 128 A6:3
- Insert:26: Eccentric_rod:3 ↔ DIN 128 A6:4
- Insert:27: DIN EN ISO 1207 M6 x 20:4 ↔ DIN 128 A6:5
- Insert:28: DIN EN ISO 1207 M6 x 20:5 ↔ DIN 128 A6:3
- Insert:29: DIN EN ISO 1207 M6 x 20:6 ↔ DIN 128 A6:4
- Insert:30: DIN EN ISO 1207 M6 x 20:1 ↔ DIN 128 A6:2
- Insert:31: DIN EN ISO 1207 M6 x 20:3 ↔ DIN 128 A6:1
- Insert:32: DIN EN ISO 1207 M6 x 20:2 ↔ DIN 128 A6:6
- Insert:33: Steam_chest_slide_value_rod_:2 ↔ DIN 934 - replaced by DIN EN 24032/28673/28674 M6:2
- Insert:34: Eccentric_rod:4 ↔ DIN 934 - replaced by DIN EN 24032/28673/28674 M6:4
- Insert:35: Eccentric_rod:3 ↔ DIN 934 - replaced by DIN EN 24032/28673/28674 M6:3
- Insert:36: Steam_chest_slide_value_rod_:1 ↔ DIN 934 - replaced by DIN EN 24032/28673/28674 M6:5
- Insert:37: Eccentric_rod:2 ↔ DIN 934 - replaced by DIN EN 24032/28673/28674 M6:1
- Insert:38: Eccentric_rod:1 ↔ DIN 934 - replaced by DIN EN 24032/28673/28674 M6:6
- Insert:39: Revert_Gear_Drag_Link_:2 ↔ DIN 128 A6:7
- Insert:40: Revert_Gear_Drag_Link_:2 ↔ DIN 128 A6:10
- Insert:41: Revert_Gear_Drag_Link_:4 ↔ DIN 128 A6:9
- Insert:42: Revert_Gear_Drag_Link_:4 ↔ DIN 128 A6:8
- Insert:43: DIN EN ISO 1207 M6 x 45:4 ↔ DIN 128 A6:10
- Insert:44: DIN EN ISO 1207 M6 x 45:3 ↔ DIN 128 A6:7
- Insert:45: DIN EN ISO 1207 M6 x 45:2 ↔ DIN 128 A6:8
- Insert:46: DIN EN ISO 1207 M6 x 45:1 ↔ DIN 128 A6:9
- Insert:47: Revert_Gear_Drag_Link_:1 ↔ DIN 934 - replaced by DIN EN 24032/28673/28674 M6:9
- Insert:48: Revert_Gear_Drag_Link_:1 ↔ DIN 934 - replaced by DIN EN 24032/28673/28674 M6:10
- Insert:49: Revert_Gear_Drag_Link_:3 ↔ DIN 934 - replaced by DIN EN 24032/28673/28674 M6:8
- Insert:50: Revert_Gear_Drag_Link_:3 ↔ DIN 934 - replaced by DIN EN 24032/28673/28674 M6:7
- Insert:51: Stand_1:1 ↔ DIN 125-1 A A 13:4
- Insert:52: Stand_1:1 ↔ DIN 125-1 A A 13:3
- Insert:53: Stand_1:1 ↔ DIN 125-1 A A 13:1
- Insert:54: Stand_1:1 ↔ DIN 125-1 A A 13:2
- Insert:55: DIN 912 - replaced by DIN EN ISO 4762 M12 x 55:1 ↔ DIN 125-1 A A 13:4
- Insert:56: DIN 912 - replaced by DIN EN ISO 4762 M12 x 55:4 ↔ DIN 125-1 A A 13:3
- Insert:57: DIN 912 - replaced by DIN EN ISO 4762 M12 x 55:3 ↔ DIN 125-1 A A 13:1
- Insert:58: DIN 912 - replaced by DIN EN ISO 4762 M12 x 55:2 ↔ DIN 125-1 A A 13:2
- Insert:59: Base:1 ↔ DIN 128 A12:2
- Insert:60: Base:1 ↔ DIN 128 A12:1
- Insert:61: Base:1 ↔ DIN 128 A12:3
- Insert:62: Base:1 ↔ DIN 128 A12:4
- Insert:63: DIN 128 A12:2 ↔ DIN 1587 M12 - SW18:1
- Insert:64: DIN 128 A12:1 ↔ DIN 1587 M12 - SW18:2
- Insert:65: DIN 128 A12:3 ↔ DIN 1587 M12 - SW18:3
- Insert:66: DIN 128 A12:4 ↔ DIN 1587 M12 - SW18:4
- Insert:67: Upper_Cylinder_Cover_26:2 ↔ DIN 128 A6:11
- Insert:68: Upper_Cylinder_Cover_26:2 ↔ DIN 128 A6:12
- Insert:69: Upper_Cylinder_Cover_26:2 ↔ DIN 128 A6:13
- Insert:70: Upper_Cylinder_Cover_26:2 ↔ DIN 128 A6:14
- Insert:71: Upper_Cylinder_Cover_26:2 ↔ DIN 128 A6:15
- Insert:72: Upper_Cylinder_Cover_26:2 ↔ DIN 128 A6:16
- Insert:73: Upper_Cylinder_Cover_26:2 ↔ DIN 128 A6:17
- Insert:74: Upper_Cylinder_Cover_26:2 ↔ DIN 128 A6:18
- Insert:75: Upper_Cylinder_Cover_26:1 ↔ DIN 128 A6:26
- Insert:76: Upper_Cylinder_Cover_26:1 ↔ DIN 128 A6:20
- Insert:77: Upper_Cylinder_Cover_26:1 ↔ DIN 128 A6:19
- Insert:78: Upper_Cylinder_Cover_26:1 ↔ DIN 128 A6:22
- Insert:79: Upper_Cylinder_Cover_26:1 ↔ DIN 128 A6:21
- Insert:80: Upper_Cylinder_Cover_26:1 ↔ DIN 128 A6:23
- Insert:81: Upper_Cylinder_Cover_26:1 ↔ DIN 128 A6:25
- Insert:82: Upper_Cylinder_Cover_26:1 ↔ DIN 128 A6:24
- Insert:83: DIN 912 - replaced by DIN EN ISO 4762 M6 x 12:11 ↔ DIN 128 A6:12
- Insert:84: DIN 912 - replaced by DIN EN ISO 4762 M6 x 12:2 ↔ DIN 128 A6:11
- Insert:85: DIN 912 - replaced by DIN EN ISO 4762 M6 x 12:1 ↔ DIN 128 A6:18
- Insert:86: DIN 912 - replaced by DIN EN ISO 4762 M6 x 12:3 ↔ DIN 128 A6:13
- Insert:87: DIN 912 - replaced by DIN EN ISO 4762 M6 x 12:12 ↔ DIN 128 A6:14
- Insert:88: DIN 912 - replaced by DIN EN ISO 4762 M6 x 12:4 ↔ DIN 128 A6:15
- Insert:89: DIN 912 - replaced by DIN EN ISO 4762 M6 x 12:10 ↔ DIN 128 A6:16
- Insert:90: DIN 912 - replaced by DIN EN ISO 4762 M6 x 12:9 ↔ DIN 128 A6:17
- Insert:91: DIN 912 - replaced by DIN EN ISO 4762 M6 x 12:5 ↔ DIN 128 A6:21
- Insert:92: DIN 912 - replaced by DIN EN ISO 4762 M6 x 12:13 ↔ DIN 128 A6:22
- Insert:93: DIN 912 - replaced by DIN EN ISO 4762 M6 x 12:6 ↔ DIN 128 A6:19
- Insert:94: DIN 912 - replaced by DIN EN ISO 4762 M6 x 12:14 ↔ DIN 128 A6:26
- Insert:95: DIN 912 - replaced by DIN EN ISO 4762 M6 x 12:7 ↔ DIN 128 A6:20
- Insert:96: DIN 912 - replaced by DIN EN ISO 4762 M6 x 12:15 ↔ DIN 128 A6:24
- Insert:97: DIN 912 - replaced by DIN EN ISO 4762 M6 x 12:16 ↔ DIN 128 A6:25
- Insert:98: DIN 912 - replaced by DIN EN ISO 4762 M6 x 12:8 ↔ DIN 128 A6:23
- Insert:99: Welding_assembly_Standard:3 ↔ DIN 128 A6:41
- Insert:100: Welding_assembly_Standard:3 ↔ DIN 128 A6:42
- Insert:101: Welding_assembly_Standard:3 ↔ DIN 128 A6:40
- Insert:102: Welding_assembly_Standard:3 ↔ DIN 128 A6:39
- Insert:103: Welding_assembly_Standard:3 ↔ DIN 128 A6:38
- Insert:104: Welding_assembly_Standard:3 ↔ DIN 128 A6:36
- Insert:105: Welding_assembly_Standard:3 ↔ DIN 128 A6:37
- Insert:106: Welding_assembly_Standard:3 ↔ DIN 128 A6:35
- Insert:107: Welding_assembly_Standard:2 ↔ DIN 128 A6:34
- Insert:108: Welding_assembly_Standard:2 ↔ DIN 128 A6:33
- Insert:109: Welding_assembly_Standard:2 ↔ DIN 128 A6:32
- Insert:110: Welding_assembly_Standard:2 ↔ DIN 128 A6:31
- Insert:111: Welding_assembly_Standard:2 ↔ DIN 128 A6:30
- Insert:112: Welding_assembly_Standard:4 ↔ DIN 128 A6:29
- Insert:113: Welding_assembly_Standard:4 ↔ DIN 128 A6:27
- Insert:114: Welding_assembly_Standard:4 ↔ DIN 128 A6:28
- Insert:115: DIN 128 A6:42 ↔ DIN 912 - replaced by DIN EN ISO 4762 M6 x 20:13
- Insert:116: DIN 128 A6:31 ↔ DIN 912 - replaced by DIN EN ISO 4762 M6 x 20:1
- Insert:117: Welding_assembly_Standard:3 ↔ DIN 128 A6:46
- Insert:118: Welding_assembly_Standard:4 ↔ DIN 128 A6:43
- Insert:119: Welding_assembly_Standard:4 ↔ DIN 128 A6:45
- Insert:120: Welding_assembly_Standard:4 ↔ DIN 128 A6:48
- Insert:121: Welding_assembly_Standard:4 ↔ DIN 128 A6:47
- Insert:122: Welding_assembly_Standard:3 ↔ DIN 128 A6:50
- Insert:123: Welding_assembly_Standard:3 ↔ DIN 128 A6:49
- Insert:124: Upper_Base_Bearing_Holder_7:2 ↔ DIN 128 A6:52
- Insert:125: Upper_Base_Bearing_Holder_7:2 ↔ DIN 128 A6:51
- Insert:126: Upper_Base_Bearing_Holder2_8:1 ↔ DIN 128 A6:54
- Insert:127: Upper_Base_Bearing_Holder2_8:1 ↔ DIN 128 A6:56
- Insert:128: Upper_Base_Bearing_Holder_7:1 ↔ DIN 128 A6:55
- Insert:129: Upper_Base_Bearing_Holder_7:1 ↔ DIN 128 A6:53
- Insert:130: DIN 933 - replaced by DIN EN 24017 M6  x 20:8 ↔ DIN 128 A6:49
- Insert:131: DIN 933 - replaced by DIN EN 24017 M6  x 20:7 ↔ DIN 128 A6:50
- Insert:132: DIN 933 - replaced by DIN EN 24017 M6  x 20:12 ↔ DIN 128 A6:48
- Insert:133: DIN 933 - replaced by DIN EN 24017 M6  x 20:14 ↔ DIN 128 A6:47
- Insert:134: DIN 933 - replaced by DIN EN 24017 M6  x 20:13 ↔ DIN 128 A6:56
- Insert:135: DIN 933 - replaced by DIN EN 24017 M6  x 20:11 ↔ DIN 128 A6:53
- Insert:136: DIN 933 - replaced by DIN EN 24017 M6  x 20:9 ↔ DIN 128 A6:52
- Insert:137: DIN 933 - replaced by DIN EN 24017 M6  x 20:10 ↔ DIN 128 A6:51
- Insert:138: DIN 933 - replaced by DIN EN 24017 M6  x 20:6 ↔ DIN 128 A6:55
- Insert:139: DIN 933 - replaced by DIN EN 24017 M6  x 20:5 ↔ DIN 128 A6:54
- Insert:140: DIN 933 - replaced by DIN EN 24017 M6  x 20:3 ↔ DIN 128 A6:46
- Insert:141: DIN 933 - replaced by DIN EN 24017 M6  x 20:2 ↔ DIN 128 A6:43
- Insert:142: DIN 933 - replaced by DIN EN 24017 M6  x 20:1 ↔ DIN 128 A6:45
- Insert:143: Welding_assembly_Standard:3 ↔ DIN 128 A6:44
- Insert:144: DIN 933 - replaced by DIN EN 24017 M6  x 20:4 ↔ DIN 128 A6:44
- Insert:145: Eccentric_rod:4 ↔ DIN 71412 A AM 6 (coned short):3
- Insert:146: Upper_Base_Bearing_Holder_7:1 ↔ DIN 71412 A AM 6 (coned short):1
- Insert:147: Eccentric_rod:3 ↔ DIN 71412 A AM 6 (coned short):4
- Insert:148: Upper_Base_Bearing_Holder2_8:1 ↔ DIN 71412 A AM 6 (coned short):2
- Insert:149: Upper_Base_Bearing_Holder_7:2 ↔ DIN 71412 A AM 6 (coned short):6
- Insert:150: Eccentric_rod:1 ↔ DIN 71412 A AM 6 (coned short):5
- Insert:151: Eccentric_rod:2 ↔ DIN 71412 A AM 6 (coned short):7
- Insert:156: Steamchest_cover_:2 ↔ DIN 128 A4:6
- Insert:157: Steamchest_cover_:2 ↔ DIN 128 A4:8
- Insert:158: Steamchest_cover_:2 ↔ DIN 128 A4:7
- Insert:159: Steamchest_cover_:2 ↔ DIN 128 A4:5
- Insert:160: DIN 912 - replaced by DIN EN ISO 4762 M4 x 35:8 ↔ DIN 128 A4:6
- Insert:161: DIN 912 - replaced by DIN EN ISO 4762 M4 x 35:7 ↔ DIN 128 A4:8
- Insert:162: DIN 912 - replaced by DIN EN ISO 4762 M4 x 35:5 ↔ DIN 128 A4:5
- Insert:163: DIN 912 - replaced by DIN EN ISO 4762 M4 x 35:6 ↔ DIN 128 A4:7
- Insert:164: DIN 912 - replaced by DIN EN ISO 4762 M4 x 35:4 ↔ DIN 128 A4:12
- Insert:165: DIN 912 - replaced by DIN EN ISO 4762 M4 x 35:3 ↔ DIN 128 A4:10
- Insert:166: DIN 912 - replaced by DIN EN ISO 4762 M4 x 35:1 ↔ DIN 128 A4:11
- Insert:167: DIN 912 - replaced by DIN EN ISO 4762 M4 x 35:2 ↔ DIN 128 A4:9
- Mate:240: Steamchest_cover_:1 ↔ DIN 912 - replaced by DIN EN ISO 4762 M4 x 35:4
- Mate:241: Steamchest_:1 ↔ Steamchest_cover_:1
- Mate:242: Steamchest_:1 ↔ DIN 912 - replaced by DIN EN ISO 4762 M4 x 35:4
- Mate:243: Steamchest_cover_:1 ↔ DIN 128 A4:12
- Mate:244: Steamchest_cover_:1 ↔ DIN 912 - replaced by DIN EN ISO 4762 M4 x 35:1
- Mate:245: Steamchest_:1 ↔ DIN 912 - replaced by DIN EN ISO 4762 M4 x 35:1
- Mate:246: Steamchest_cover_:1 ↔ DIN 128 A4:11
- Insert:168: Steamchest_cover_:1 ↔ DIN 128 A4:9
- Mate:247: Steamchest_cover_:1 ↔ DIN 128 A4:10
- Mate:248: Assembly_Eccentric:1 ↔ DIN 916 M4  x  5:5
- Flush:12 (-1 mm): Assembly_Eccentric:1 ↔ DIN 916 M4  x  5:5
- Insert:169: Revert_gear_level_link_pt:1 ↔ DIN 916 M4  x  5:3
- Insert:170: Reverse_gear_lever_:1 ↔ DIN 916 M4  x  5:6
- Insert:171: Reverse_gear_lever_:1 ↔ DIN 916 M4  x  5:4
- Insert:172: Revert_gear_level_link_pt:2 ↔ DIN 916 M4  x  5:2
- Mate:249: Assembly_Eccentric:2 ↔ DIN 916 M4  x  5:1
- Flush:13 (-1 mm): Assembly_Eccentric:2 ↔ DIN 916 M4  x  5:1
